# Autodesk Inventor assembly: NASA-20-FR
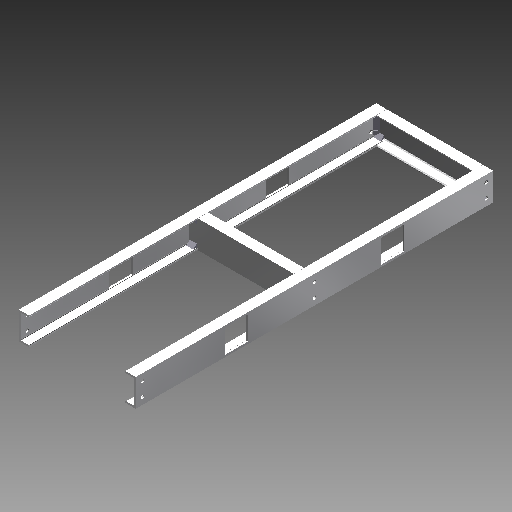
[picture p0: Inventor's stored thumbnail of the model, 512x512]
Saved by Autodesk Inventor 2019 (Build 230136000, 136)
## iProperties
Created: 2019-09-07
Part Number: NASA-20-FR
Document SubType Name: Weldment
Designer: Rick Szalay
Weld Material: Welded Aluminum-6061
Author: Rick Szalay
## Documents named in this file (4)
- C:\Users\Rick Szalay\Documents\Inventor\NASA 20\NASA-20\FR\NASA-20-FR.iam
- C:\Users\Rick Szalay\Documents\Inventor\NASA 20\NASA-20\FR\NASA-20-FR-SP-01.ipt
- C:\Users\Rick Szalay\Documents\Inventor\NASA 20\NASA-20\FR\NASA-20-FR-BK-01.ipt
- C:\Users\Rick Szalay\Documents\Inventor\NASA 20\NASA-20\FR\NASA-20-FR-FP-01.ipt
## Components (4 placed, 3 different names)
1. NASA-20-FR-SP-01:1 — Mate:3, Mate:4
2. NASA-20-FR-SP-01:2 — Mate:3
3. NASA-20-FR-BK-01:1 — Flush:7
4. NASA-20-FR-FP-01:1 — Flush:6
## Relationships (11: Flush 7, Mate 4)
- [Flush]: NASA-20-FR-SP-01:1 ↔ NASA-20-FR-SP-01:2
- [Flush]: NASA-20-FR-SP-01:1 ↔ NASA-20-FR-SP-01:2
- [Flush]: NASA-20-FR-SP-01:1 ↔ NASA-20-FR-BK-01:1
- [Flush]: NASA-20-FR-SP-01:1 ↔ NASA-20-FR-BK-01:1
- [Mate]: NASA-20-FR-SP-01:1 ↔ NASA-20-FR-BK-01:1
- [Mate]: NASA-20-FR-SP-01:1 ↔ NASA-20-FR-FP-01:1
- [Flush]: NASA-20-FR-SP-01:1 ↔ NASA-20-FR-FP-01:1
- Flush:6 (19.05 mm): NASA-20-FR-FP-01:1
- Mate:3 (-215.9 mm): NASA-20-FR-SP-01:1 ↔ NASA-20-FR-SP-01:2
- Mate:4: NASA-20-FR-SP-01:1
- Flush:7: NASA-20-FR-BK-01:1
## Named parameters: Width = 215.9 mm, Length = 660.4 mm
